# Autodesk Inventor assembly: XCarriage
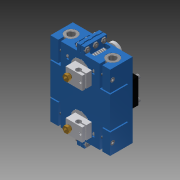
[picture p0: Inventor's stored thumbnail of the model, 180x180]
Saved by Autodesk Inventor 2015 (Build 190159000, 159)
## iProperties
Created: 2014-08-22
Part Number: XCarriage
Document SubType Name: Assembly
Designer: t_clevj
Author: t_clevj
## Documents named in this file (12)
- C:\Users\Jack\ownCloud\Projects\CoreXY\InventorModel\XAxis\DualE3DXEnd\XCarriage.iam
- C:\Users\Jack\ownCloud\Projects\CoreXY\InventorModel\XAxis\DualE3DXEnd\XCarriageBeltClampRight.ipt
- C:\Users\Jack\ownCloud\Projects\CoreXY\InventorModel\XAxis\DualE3DXEnd\XCarriageV9.ipt
- C:\Users\Jack\ownCloud\Projects\CoreXY\InventorModel\XAxis\DualE3DXEnd\XCarriageV9Top.ipt
- C:\Users\Jack\ownCloud\Projects\CoreXY\InventorModel\HotEnds\E3DV6\E3DV6.iam
- C:\Users\Jack\ownCloud\Projects\CoreXY\InventorModel\Electronics\Fan30mm.ipt
- C:\Users\Jack\ownCloud\Projects\CoreXY\InventorModel\XAxis\DualE3DXEnd\XCarriageBeltClampLeft.ipt
- C:\Users\Jack\ownCloud\Projects\CoreXY\InventorModel\Hardware\Bolts\SHCS\SHCS3\SHCS3x20.ipt
- C:\Users\Jack\ownCloud\Projects\CoreXY\InventorModel\Hardware\Bolts\SHCS\SHCS3\SHCS3x10.ipt
- C:\Users\Jack\ownCloud\Projects\CoreXY\InventorModel\Hardware\Nuts\Nut3.ipt
- C:\Users\Jack\ownCloud\Projects\CoreXY\InventorModel\Hardware\Bolts\SHCS\SHCS3\SHCS3x14.ipt
- C:\Users\Jack\ownCloud\Projects\CoreXY\InventorModel\Hardware\Bearing\BearingLinear\BearingLinearLMU8.ipt
## Components (48 placed, 11 different names)
1. XCarriageBeltClampRight:1 — Mate:4, Mate:5, Mate:6, Mate:33, Mate:34, Mate:35, Mate:36, Mate:37, Mate:38
2. XCarriageV9:1 — Mate:1, Mate:2, Mate:3, Mate:4, Mate:5, Mate:6, Angle:1, Angle:2, Mate:22, Mate:23, Mate:24, Mate:25, Mate:26, Mate:27, Mate:28, Mate:29, Mate:30, Mate:31, Mate:32, Mate:51, Mate:52, Mate:53, Mate:54, Mate:55, Mate:56, Angle:3, Angle:4, Angle:5, Angle:6, Angle:7, Angle:8, Mate:61, Mate:62, Mate:63, Mate:64, Angle:9, Angle:10, Angle:11, Angle:12, Mate:65, Mate:66, Mate:70, Mate:71, Mate:72, Angle:13, Angle:14, Angle:15, Angle:16, Mate:97, Mate:98, Mate:99, Mate:100, Flush:3, Flush:4, Flush:5, Flush:6, Mate:101, Mate:102, Mate:103
3. XCarriageV9Top:1 — Mate:1, Mate:2, Mate:3, Mate:10, Mate:11, Flush:1, Flush:2, Mate:12, Mate:13, Mate:14, Mate:15, Mate:16, Mate:17, Mate:67, Mate:68, Mate:69, Mate:93, Mate:94, Mate:95, Mate:96, Angle:17, Angle:18, Angle:19, Angle:20
4. E3DV6:1 [sub-assembly] — Mate:10, Flush:1, Angle:2
5. E3DV6:2 [sub-assembly] — Mate:11, Flush:2, Angle:1
6. Fan30mm:1 — Mate:13, Mate:14, Mate:15, Mate:75, Mate:76, Mate:77, Mate:78, Mate:83, Mate:84, Mate:85, Mate:87
7. Fan30mm:2 — Mate:12, Mate:16, Mate:17, Mate:73, Mate:74, Mate:79, Mate:80, Mate:81, Mate:82, Mate:86, Mate:88
8. XCarriageBeltClampLeft:1 — Mate:22, Mate:23, Mate:24, Mate:39, Mate:40, Mate:41, Mate:42, Mate:43, Mate:44
9. BearingLinearLMU8:1 — Mate:99, Flush:5
10. BearingLinearLMU8:2 — Mate:98, Flush:3
11. BearingLinearLMU8:3 — Mate:97, Flush:6
12. BearingLinearLMU8:4 — Mate:100, Flush:4
13. SHCS3x10:4 — Mate:33, Mate:38, Mate:45
14. SHCS3x10:1 — Mate:34, Mate:37, Mate:46
15. SHCS3x10:5 — Mate:35, Mate:36, Mate:47
16. Nut3:4 — Mate:47, Mate:52, Angle:8
17. Nut3:2 — Mate:46, Mate:53, Angle:7
18. Nut3:1 — Mate:45, Mate:54, Angle:6
19. SHCS3x10:2 — Mate:41, Mate:42, Mate:48
20. SHCS3x10:3 — Mate:40, Mate:43, Mate:49
21. SHCS3x10:6 — Mate:39, Mate:44, Mate:50
22. Nut3:3 — Mate:48, Mate:55, Angle:3
23. Nut3:10 — Mate:49, Mate:56, Angle:4
24. Nut3:8 — Mate:50, Mate:51, Angle:5
25. SHCS3x20:2 — Mate:26, Mate:32, Mate:58
26. SHCS3x20:1 — Mate:25, Mate:31, Mate:57
27. SHCS3x20:3 — Mate:28, Mate:30, Mate:59
28. SHCS3x20:4 — Mate:27, Mate:29, Mate:60
29. Nut3:9 — Mate:59, Mate:62, Angle:11
30. Nut3:5 — Mate:57, Mate:63, Angle:10
31. Nut3:6 — Mate:58, Mate:64, Angle:9
32. Nut3:7 — Mate:60, Mate:61, Angle:12
33. Nut3:13 — Mate:68, Mate:71, Angle:15
34. Nut3:11 — Mate:65, Mate:66, Angle:14
35. Nut3:15 — Mate:92, Mate:96, Angle:17
36. Nut3:16 — Mate:91, Mate:95, Angle:18
37. Nut3:14 — Mate:69, Mate:70, Angle:16
38. Nut3:18 — Mate:89, Mate:93, Angle:19
39. Nut3:17 — Mate:90, Mate:94, Angle:20
40. Nut3:12 — Mate:67, Mate:72, Angle:13
41. SHCS3x20:8 — Mate:73, Mate:80
42. SHCS3x14:1 — Mate:81, Mate:88, Mate:92
43. SHCS3x14:3 — Mate:83, Mate:87, Mate:91
44. SHCS3x14:4 — Mate:84, Mate:85, Mate:89
45. SHCS3x14:2 — Mate:82, Mate:86, Mate:90
46. SHCS3x20:6 — Mate:74, Mate:79
47. SHCS3x20:7 — Mate:76, Mate:77
48. SHCS3x20:5 — Mate:75, Mate:78
## Relationships (122: Mate 96, Angle 20, Flush 6)
- Mate:1: XCarriageV9:1 ↔ XCarriageV9Top:1
- Mate:2: XCarriageV9:1 ↔ XCarriageV9Top:1
- Mate:3: XCarriageV9:1 ↔ XCarriageV9Top:1
- Mate:4: XCarriageBeltClampRight:1 ↔ XCarriageV9:1
- Mate:5: XCarriageBeltClampRight:1 ↔ XCarriageV9:1
- Mate:6 (1 mm): XCarriageBeltClampRight:1 ↔ XCarriageV9:1
- Mate:10: XCarriageV9Top:1 ↔ E3DV6:1
- Mate:11: XCarriageV9Top:1 ↔ E3DV6:2
- Flush:1 (-1 mm): XCarriageV9Top:1 ↔ E3DV6:1
- Flush:2 (-1 mm): XCarriageV9Top:1 ↔ E3DV6:2
- Angle:1 (0 deg): XCarriageV9:1 ↔ E3DV6:2
- Angle:2 (0 deg): XCarriageV9:1 ↔ E3DV6:1
- Mate:12: XCarriageV9Top:1 ↔ Fan30mm:2
- Mate:13: XCarriageV9Top:1 ↔ Fan30mm:1
- Mate:14: XCarriageV9Top:1 ↔ Fan30mm:1
- Mate:15: XCarriageV9Top:1 ↔ Fan30mm:1
- Mate:16: XCarriageV9Top:1 ↔ Fan30mm:2
- Mate:17: XCarriageV9Top:1 ↔ Fan30mm:2
- Mate:22 (1 mm): XCarriageV9:1 ↔ XCarriageBeltClampLeft:1
- Mate:23: XCarriageV9:1 ↔ XCarriageBeltClampLeft:1
- Mate:24: XCarriageV9:1 ↔ XCarriageBeltClampLeft:1
- Mate:25: XCarriageV9:1 ↔ SHCS3x20:1
- Mate:26: XCarriageV9:1 ↔ SHCS3x20:2
- Mate:27: XCarriageV9:1 ↔ SHCS3x20:4
- Mate:28: XCarriageV9:1 ↔ SHCS3x20:3
- Mate:29: XCarriageV9:1 ↔ SHCS3x20:4
- Mate:30: XCarriageV9:1 ↔ SHCS3x20:3
- Mate:31: XCarriageV9:1 ↔ SHCS3x20:1
- Mate:32: XCarriageV9:1 ↔ SHCS3x20:2
- Mate:33: XCarriageBeltClampRight:1 ↔ SHCS3x10:4
- Mate:34: XCarriageBeltClampRight:1 ↔ SHCS3x10:1
- Mate:35: XCarriageBeltClampRight:1 ↔ SHCS3x10:5
- Mate:36: XCarriageBeltClampRight:1 ↔ SHCS3x10:5
- Mate:37: XCarriageBeltClampRight:1 ↔ SHCS3x10:1
- Mate:38: XCarriageBeltClampRight:1 ↔ SHCS3x10:4
- Mate:39: XCarriageBeltClampLeft:1 ↔ SHCS3x10:6
- Mate:40: XCarriageBeltClampLeft:1 ↔ SHCS3x10:3
- Mate:41: XCarriageBeltClampLeft:1 ↔ SHCS3x10:2
- Mate:42: XCarriageBeltClampLeft:1 ↔ SHCS3x10:2
- Mate:43: XCarriageBeltClampLeft:1 ↔ SHCS3x10:3
- Mate:44: XCarriageBeltClampLeft:1 ↔ SHCS3x10:6
- Mate:45: SHCS3x10:4 ↔ Nut3:1
- Mate:46: SHCS3x10:1 ↔ Nut3:2
- Mate:47: SHCS3x10:5 ↔ Nut3:4
- Mate:48: SHCS3x10:2 ↔ Nut3:3
- Mate:49: SHCS3x10:3 ↔ Nut3:10
- Mate:50: SHCS3x10:6 ↔ Nut3:8
- Mate:51: XCarriageV9:1 ↔ Nut3:8
- Mate:52: XCarriageV9:1 ↔ Nut3:4
- Mate:53: XCarriageV9:1 ↔ Nut3:2
- Mate:54: XCarriageV9:1 ↔ Nut3:1
- Mate:55: XCarriageV9:1 ↔ Nut3:3
- Mate:56: XCarriageV9:1 ↔ Nut3:10
- Angle:3 (0 deg): XCarriageV9:1 ↔ Nut3:3
- Angle:4 (0 deg): XCarriageV9:1 ↔ Nut3:10
- Angle:5 (0 deg): XCarriageV9:1 ↔ Nut3:8
- Angle:6 (0 deg): XCarriageV9:1 ↔ Nut3:1
- Angle:7 (0 deg): XCarriageV9:1 ↔ Nut3:2
- Angle:8 (0 deg): XCarriageV9:1 ↔ Nut3:4
- Mate:57: SHCS3x20:1 ↔ Nut3:5
- Mate:58: SHCS3x20:2 ↔ Nut3:6
- Mate:59: SHCS3x20:3 ↔ Nut3:9
- Mate:60: SHCS3x20:4 ↔ Nut3:7
- Mate:61: XCarriageV9:1 ↔ Nut3:7
- Mate:62: XCarriageV9:1 ↔ Nut3:9
- Mate:63: XCarriageV9:1 ↔ Nut3:5
- Mate:64: XCarriageV9:1 ↔ Nut3:6
- Angle:9 (0 deg): XCarriageV9:1 ↔ Nut3:6
- Angle:10 (0 deg): XCarriageV9:1 ↔ Nut3:5
- Angle:11 (0 deg): XCarriageV9:1 ↔ Nut3:9
- Angle:12 (0 deg): XCarriageV9:1 ↔ Nut3:7
- Mate:65: XCarriageV9:1 ↔ Nut3:11
- Mate:66: XCarriageV9:1 ↔ Nut3:11
- Mate:67: XCarriageV9Top:1 ↔ Nut3:12
- Mate:68: XCarriageV9Top:1 ↔ Nut3:13
- Mate:69: XCarriageV9Top:1 ↔ Nut3:14
- Mate:70: XCarriageV9:1 ↔ Nut3:14
- Mate:71: XCarriageV9:1 ↔ Nut3:13
- Mate:72: XCarriageV9:1 ↔ Nut3:12
- Angle:13 (0 deg): XCarriageV9:1 ↔ Nut3:12
- Angle:14 (0 deg): XCarriageV9:1 ↔ Nut3:11
- Angle:15 (0 deg): XCarriageV9:1 ↔ Nut3:13
- Angle:16 (0 deg): XCarriageV9:1 ↔ Nut3:14
- Mate:73: Fan30mm:2 ↔ SHCS3x20:8
- Mate:74: Fan30mm:2 ↔ SHCS3x20:6
- Mate:75: Fan30mm:1 ↔ SHCS3x20:5
- Mate:76: Fan30mm:1 ↔ SHCS3x20:7
- Mate:77: Fan30mm:1 ↔ SHCS3x20:7
- Mate:78: Fan30mm:1 ↔ SHCS3x20:5
- Mate:79: Fan30mm:2 ↔ SHCS3x20:6
- Mate:80: Fan30mm:2 ↔ SHCS3x20:8
- Mate:81: Fan30mm:2 ↔ SHCS3x14:1
- Mate:82: Fan30mm:2 ↔ SHCS3x14:2
- Mate:83: Fan30mm:1 ↔ SHCS3x14:3
- Mate:84: Fan30mm:1 ↔ SHCS3x14:4
- Mate:85: Fan30mm:1 ↔ SHCS3x14:4
- Mate:86: Fan30mm:2 ↔ SHCS3x14:2
- Mate:87: Fan30mm:1 ↔ SHCS3x14:3
- Mate:88: Fan30mm:2 ↔ SHCS3x14:1
- Mate:89: Nut3:18 ↔ SHCS3x14:4
- Mate:90: Nut3:17 ↔ SHCS3x14:2
- Mate:91: Nut3:16 ↔ SHCS3x14:3
- Mate:92: Nut3:15 ↔ SHCS3x14:1
- Mate:93: XCarriageV9Top:1 ↔ Nut3:18
- Mate:94: XCarriageV9Top:1 ↔ Nut3:17
- Mate:95: XCarriageV9Top:1 ↔ Nut3:16
- Mate:96: XCarriageV9Top:1 ↔ Nut3:15
- Angle:17 (0 deg): XCarriageV9Top:1 ↔ Nut3:15
- Angle:18 (0 deg): XCarriageV9Top:1 ↔ Nut3:16
- Angle:19 (0 deg): XCarriageV9Top:1 ↔ Nut3:18
- Angle:20 (0 deg): XCarriageV9Top:1 ↔ Nut3:17
- Mate:97: XCarriageV9:1 ↔ BearingLinearLMU8:3
- Mate:98: XCarriageV9:1 ↔ BearingLinearLMU8:2
- Mate:99: XCarriageV9:1 ↔ BearingLinearLMU8:1
- Mate:100: XCarriageV9:1 ↔ BearingLinearLMU8:4
- Flush:3: XCarriageV9:1 ↔ BearingLinearLMU8:2
- Flush:4: XCarriageV9:1 ↔ BearingLinearLMU8:4
- Flush:5: XCarriageV9:1 ↔ BearingLinearLMU8:1
- Flush:6: XCarriageV9:1 ↔ BearingLinearLMU8:3
- Mate:101: XCarriageV9:1
- Mate:102: XCarriageV9:1
- Mate:103: XCarriageV9:1
